# Autodesk Inventor assembly: LAMP_OUTDOOR_BATTERY
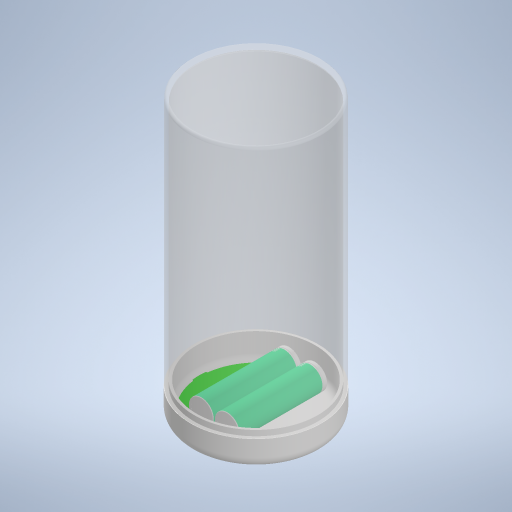
[picture p0: Inventor's stored thumbnail of the model, 512x512]
Saved by Autodesk Inventor 2024 (Build 280153000, 153)
## iProperties
Created: 2025-01-19
Part Number: LAMP_OUTDOOR_BATTERY
Document SubType Name: Assembly
Designer: malam
Author: malam
## Documents named in this file (5)
- C:\Users\malam\Documents\6 - PROJET\15 - LAMP OUTDOOR BATTERY\LAMP-OUTDOOR-BATTERY\2 - CONCEPTION 3D\20 - CONCEPTION 3D\LAMP_OUTDOOR_BATTERY.iam
- C:\Users\malam\Documents\6 - PROJET\15 - LAMP OUTDOOR BATTERY\LAMP-OUTDOOR-BATTERY\2 - CONCEPTION 3D\20 - CONCEPTION 3D\Socle test mesure.ipt
- C:\Users\malam\Documents\6 - PROJET\15 - LAMP OUTDOOR BATTERY\LAMP-OUTDOOR-BATTERY\2 - CONCEPTION 3D\20 - CONCEPTION 3D\18650Battery.ipt
- C:\Users\malam\Documents\6 - PROJET\15 - LAMP OUTDOOR BATTERY\LAMP-OUTDOOR-BATTERY\2 - CONCEPTION 3D\20 - CONCEPTION 3D\Test_PCB.ipt
- C:\Users\malam\Documents\6 - PROJET\15 - LAMP OUTDOOR BATTERY\LAMP-OUTDOOR-BATTERY\2 - CONCEPTION 3D\20 - CONCEPTION 3D\Bocal.ipt
## Components (5 placed, 4 different names)
1. Socle test mesure:1 — Affleurement:5, Placage:1, Placage:2
2. 18650Battery:2 — Affleurement:2, Tangente:1, Affleurement:4, Affleurement:5
3. 18650Battery:3 — Affleurement:2, Tangente:1, Affleurement:4
4. Test_PCB:1
5. Bocal:1 — Placage:1, Placage:2
## Relationships (6: Flush 3, Mate 2, Tangent 1)
- Affleurement:2 [Flush]: 18650Battery:2 ↔ 18650Battery:3
- Tangente:1 (1 mm): 18650Battery:2 ↔ 18650Battery:3
- Affleurement:4 [Flush]: 18650Battery:2 ↔ 18650Battery:3
- Affleurement:5 [Flush]: Socle test mesure:1 ↔ 18650Battery:2
- Placage:1 [Mate]: Socle test mesure:1 ↔ Bocal:1
- Placage:2 [Mate]: Socle test mesure:1 ↔ Bocal:1
